# Autodesk Inventor assembly: Assembly
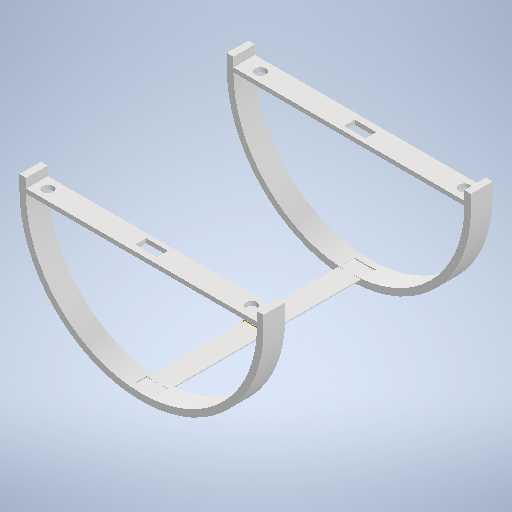
[picture p0: Inventor's stored thumbnail of the model, 512x512]
Saved by Autodesk Inventor 2025 (Build 290162010, 162A)
## iProperties
Created: 2024-06-06
Part Number: Assembly
Document SubType Name: Assembly
Designer: vncnt
Author: vncnt
## Documents named in this file (3)
- C:\Users\vncnt\Downloads\Assembly.iam
- C:\Users\vncnt\Downloads\Siding.ipt
- C:\Users\vncnt\Downloads\Lock.ipt
## Components (3 placed, 2 different names)
1. Siding:1 — Mate:1, Tangent:1
2. Siding:2
3. Lock:1 — Mate:1, Tangent:1
## Relationships (2: Mate 1, Tangent 1)
- Mate:1: Siding:1 ↔ Lock:1
- Tangent:1: Siding:1 ↔ Lock:1
